# Autodesk Inventor assembly: EnsamblajeLampara
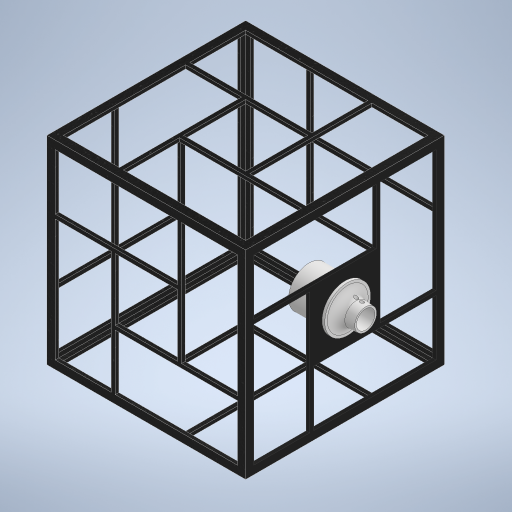
[picture p0: Inventor's stored thumbnail of the model, 512x512]
Saved by Autodesk Inventor 2024 (Build 280153000, 153)
## iProperties
Created: 2023-12-01
Part Number: EnsamblajeLampara
Document SubType Name: Assembly
Designer: sergi
Author: sergi
## Documents named in this file (5)
- C:\Users\sergi\OneDrive\Escritorio\Projects\07. Home\Kumiko lamp\Inventor\EnsamblajeLampara.iam
- C:\Users\sergi\OneDrive\Escritorio\Projects\07. Home\Kumiko lamp\Inventor\Lampara2.ipt
- C:\Users\sergi\OneDrive\Escritorio\Projects\07. Home\Kumiko lamp\Inventor\Lampara2base.ipt
- C:\Users\sergi\OneDrive\Escritorio\Projects\07. Home\Kumiko lamp\Inventor\Bombilla.ipt
- C:\Users\sergi\OneDrive\Escritorio\Projects\07. Home\Kumiko lamp\Inventor\SoporteBombilla.ipt
## Components (8 placed, 4 different names)
1. Lampara2:1 — Coincidencia:1, Coincidencia:2, Coincidencia:6, Coincidencia:7, Coincidencia:8, Coincidencia:9, Coincidencia:12
2. Lampara2:2 — Coincidencia:1, Coincidencia:3, Coincidencia:4, Coincidencia:5, Coincidencia:6, Coincidencia:7, Coincidencia:13, Coincidencia:16
3. Lampara2:3 — Coincidencia:2, Coincidencia:8, Coincidencia:9, Coincidencia:11
4. Lampara2:4 — Coincidencia:3, Coincidencia:4, Coincidencia:5, Coincidencia:10, Coincidencia:14, Coincidencia:15
5. Lampara2:5 — Coincidencia:10, Coincidencia:11, Coincidencia:15, Coincidencia:16
6. Lampara2base:1 — Coincidencia:12, Coincidencia:13, Coincidencia:14, Coincidencia:18, Coincidencia:19
7. Bombilla:1 — Coincidencia:17, Coincidencia:20
8. SoporteBombilla:1 — Coincidencia:17, Coincidencia:18, Coincidencia:19, Coincidencia:20
## Relationships (20: Mate 20)
- Coincidencia:1 [Mate]: Lampara2:1 ↔ Lampara2:2
- Coincidencia:2 [Mate]: Lampara2:1 ↔ Lampara2:3
- Coincidencia:3 [Mate]: Lampara2:2 ↔ Lampara2:4
- Coincidencia:4 [Mate]: Lampara2:2 ↔ Lampara2:4
- Coincidencia:5 [Mate]: Lampara2:2 ↔ Lampara2:4
- Coincidencia:6 [Mate]: Lampara2:1 ↔ Lampara2:2
- Coincidencia:7 [Mate]: Lampara2:1 ↔ Lampara2:2
- Coincidencia:8 [Mate]: Lampara2:1 ↔ Lampara2:3
- Coincidencia:9 [Mate]: Lampara2:1 ↔ Lampara2:3
- Coincidencia:10 [Mate]: Lampara2:4 ↔ Lampara2:5
- Coincidencia:11 [Mate]: Lampara2:3 ↔ Lampara2:5
- Coincidencia:12 [Mate]: Lampara2:1 ↔ Lampara2base:1
- Coincidencia:13 [Mate]: Lampara2:2 ↔ Lampara2base:1
- Coincidencia:14 [Mate]: Lampara2:4 ↔ Lampara2base:1
- Coincidencia:15 [Mate]: Lampara2:4 ↔ Lampara2:5
- Coincidencia:16 [Mate]: Lampara2:2 ↔ Lampara2:5
- Coincidencia:17 [Mate]: Bombilla:1 ↔ SoporteBombilla:1
- Coincidencia:18 [Mate]: Lampara2base:1 ↔ SoporteBombilla:1
- Coincidencia:19 [Mate]: Lampara2base:1 ↔ SoporteBombilla:1
- Coincidencia:20 [Mate]: Bombilla:1 ↔ SoporteBombilla:1
